# Autodesk Inventor assembly: Vex Traction Wheel 6x2
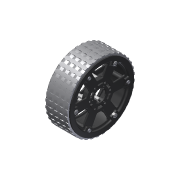
[picture p0: Inventor's stored thumbnail of the model, 180x180]
Saved by Autodesk Inventor 2013 (Build 170138000, 138)
## iProperties
Created: 2012-12-09
Part Number: Vex Traction Wheel 6x2
Document SubType Name: Assembly
Designer: Nemo
Author: Nemo
## Documents named in this file (7)
- H:\Nemo\Documents\Robotics\COTS Parts\Wheels\VexPro Traction Wheels\Vex Traction Wheel 6x2.iam
- H:\Nemo\Documents\Robotics\COTS Parts\Wheels\VexPro Traction Wheels\Components\Traction Wheel Body 6in.ipt
- H:\Nemo\Documents\Robotics\COTS Parts\Fasteners\8-32 locknut.ipt
- H:\Nemo\Documents\Robotics\COTS Parts\Wheels\VexPro Traction Wheels\Components\Traction Wheel extension 6in.ipt
- H:\Nemo\Documents\Robotics\COTS Parts\Fasteners\Hex Standoff 8-32 x1750.ipt
- H:\Nemo\Documents\Robotics\COTS Parts\Fasteners\8-32 SHCS x2250.ipt
- H:\Nemo\Documents\Robotics\COTS Parts\Wheels\VexPro Traction Wheels\Components\6 in Traction Tire.iam
## Components (26 placed, 6 different names)
1. Traction Wheel Body 6in:1 — Mate:1, Mate:2, Angle:1, Insert:1, Insert:2, Angle:2, Mate:6, Mate:10, Mate:12, Insert:6
2. Traction Wheel Body 6in:2 — Mate:3, Mate:4, Angle:3, Insert:5, Mate:8, Insert:7, Mate:15
3. Traction Wheel extension 6in:1 — Mate:5, Mate:6, Mate:8, Flush:1, Mate:11
4. Traction Wheel extension 6in:2 — Mate:9, Mate:10, Mate:11, Mate:12
5. 6 in Traction Tire:1 [sub-assembly] — Mate:13, Mate:14, Mate:15, Mate:18
6. 6 in Traction Tire:2 [sub-assembly] — Mate:16, Mate:17, Mate:18, Mate:21
7. 6 in Traction Tire:3 [sub-assembly] — Mate:19, Mate:20, Mate:21, Mate:24
8. 6 in Traction Tire:4 [sub-assembly] — Mate:22, Mate:23, Mate:24
9. Hex Standoff 8-32 x1750:1 — Angle:1, Insert:1
10. Hex Standoff 8-32 x1750:2
11. Hex Standoff 8-32 x1750:3
12. Hex Standoff 8-32 x1750:4
13. Hex Standoff 8-32 x1750:5
14. Hex Standoff 8-32 x1750:6
15. 8-32 SHCS x2250:2 — Insert:6
16. 8-32 locknut:2 — Angle:3, Insert:5
17. 8-32 SHCS x2250:1 — Insert:7
18. 8-32 locknut:1 — Insert:2, Angle:2
19. 8-32 SHCS x2250:3
20. 8-32 locknut:3
21. 8-32 SHCS x2250:4
22. 8-32 locknut:4
23. 8-32 SHCS x2250:5
24. 8-32 locknut:5
25. 8-32 SHCS x2250:6
26. 8-32 locknut:6
## Component patterns: (6 elements, first: Hex Standoff 8-32 x1750:1), (3 elements, first: 8-32 SHCS x2250:2 + 8-32 locknut:2 + 8-32 SHCS x2250:1 + 8-32 locknut:1)
## Relationships (32: Mate 23, Insert 5, Angle 3, Flush 1)
- Mate:1: Traction Wheel Body 6in:1
- Mate:2: Traction Wheel Body 6in:1
- Angle:1 (0 deg): Traction Wheel Body 6in:1 ↔ Hex Standoff 8-32 x1750:1
- Insert:1: Traction Wheel Body 6in:1 ↔ Hex Standoff 8-32 x1750:1
- Insert:2: Traction Wheel Body 6in:1 ↔ 8-32 locknut:1
- Angle:2 (0 deg): Traction Wheel Body 6in:1 ↔ 8-32 locknut:1
- Mate:3: Traction Wheel Body 6in:2
- Mate:4: Traction Wheel Body 6in:2
- Angle:3 (0 deg): Traction Wheel Body 6in:2 ↔ 8-32 locknut:2
- Insert:5: Traction Wheel Body 6in:2 ↔ 8-32 locknut:2
- Mate:5: Traction Wheel extension 6in:1
- Mate:6: Traction Wheel Body 6in:1 ↔ Traction Wheel extension 6in:1
- Mate:8: Traction Wheel Body 6in:2 ↔ Traction Wheel extension 6in:1
- Flush:1: Traction Wheel extension 6in:1
- Mate:9: Traction Wheel extension 6in:2
- Mate:10: Traction Wheel Body 6in:1 ↔ Traction Wheel extension 6in:2
- Mate:11: Traction Wheel extension 6in:1 ↔ Traction Wheel extension 6in:2
- Mate:12: Traction Wheel Body 6in:1 ↔ Traction Wheel extension 6in:2
- Insert:6: Traction Wheel Body 6in:1 ↔ 8-32 SHCS x2250:2
- Insert:7: Traction Wheel Body 6in:2 ↔ 8-32 SHCS x2250:1
- Mate:13: 6 in Traction Tire:1
- Mate:14: 6 in Traction Tire:1
- Mate:15: Traction Wheel Body 6in:2 ↔ 6 in Traction Tire:1
- Mate:16: 6 in Traction Tire:2
- Mate:17: 6 in Traction Tire:2
- Mate:18: 6 in Traction Tire:1 ↔ 6 in Traction Tire:2
- Mate:19: 6 in Traction Tire:3
- Mate:20: 6 in Traction Tire:3
- Mate:21: 6 in Traction Tire:2 ↔ 6 in Traction Tire:3
- Mate:22: 6 in Traction Tire:4
- Mate:23: 6 in Traction Tire:4
- Mate:24: 6 in Traction Tire:3 ↔ 6 in Traction Tire:4
